# Autodesk Inventor assembly: KONARM_CALY
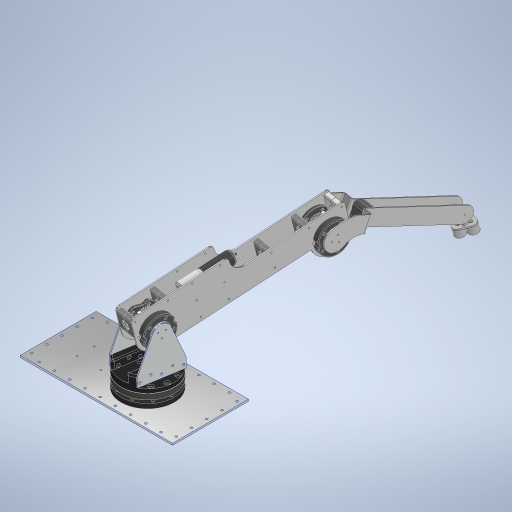
[picture p0: Inventor's stored thumbnail of the model, 512x512]
Saved by Autodesk Inventor 2023 (Build 270158000, 158)
## iProperties
Created: 2023-01-29
Part Number: KONARM_CALY
Document SubType Name: Assembly
Designer: Kamil
Mass: 3739.02 g
Surface Area: 9840.59 cm^2
Volume: 2452.75 cm^3
Density: 1.52442 g/cm^3
Author: Kamil
## Documents named in this file (4)
- D:\KONARM\KONARM_CALY.iam
- D:\KONARM\konarm 3 przegub\Konarm_3_przegub_v2.iam
- D:\KONARM\Konarm_1_przegub_final\I_Przegub_final.iam
- C:\Users\Kamil\Documents\Inventor\Konarm\Łącznik.ipt
## Components (3 placed, 3 different names)
1. Konarm_3_przegub_v2:2 [sub-assembly] — Zestawiające:1, Zestawiające:3, Zestawiające:4, Zestawiające:5
2. Łącznik:1 — Równoległe:1
3. I_Przegub_final:1 [sub-assembly] — Równoległe:1, Zestawiające:1, Zestawiające:3, Zestawiające:4, Zestawiające:5
## Relationships (5: Mate 4, Flush 1)
- Równoległe:1 [Flush]: Łącznik:1 ↔ I_Przegub_final:1
- Zestawiające:1 [Mate]: Konarm_3_przegub_v2:2 ↔ I_Przegub_final:1
- Zestawiające:3 [Mate]: Konarm_3_przegub_v2:2 ↔ I_Przegub_final:1
- Zestawiające:4 [Mate]: Konarm_3_przegub_v2:2 ↔ I_Przegub_final:1
- Zestawiające:5 [Mate]: Konarm_3_przegub_v2:2 ↔ I_Przegub_final:1
